# Autodesk Inventor assembly: BG200_trajan20_21
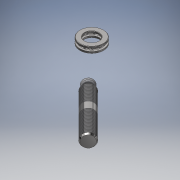
[picture p0: Inventor's stored thumbnail of the model, 180x180]
Saved by Autodesk Inventor 2022.2 (Build 262287000, 287)
## iProperties
Company: HTBLA Kaindorf
RuleStatus: InUse
Created: 2022-08-02
Part Number: BG200_trajan20_21
Project: Zeichenmaschine_v2
Material: Generisch
Description: rolle
Document SubType Name: Assembly
Designer: trajan20
AfterDocNew0: iProperties-Editor_aufrufen
Author: jan
Keywords: 2021
## Documents named in this file (5)
- C:\Users\jan\Documents\DrawMachine\DrawMachineConstruction\Projekt\Zeichenmaschine_v2\BG200_trajan20_21_Zeichenmaschine_v2_rolle.iam
- C:\Users\jan\Documents\DrawMachine\DrawMachineConstruction\Projekt\Zeichenmaschine_v2\BT105_trajan20_21_Zeichenmaschine_v2_halter final.ipt
- C:\Users\jan\Documents\DrawMachine\DrawMachineConstruction\Projekt\Zeichenmaschine_v2\BT101_trajan20_21_Zeichenmaschine_v2_rad.ipt
- C:\Users\jan\Documents\DrawMachine\DrawMachineConstruction\Projekt\Zeichenmaschine_v2\BG200_trajan20_21_Zeichenmaschine_v2_rolle\Konstruktions-Assistent\Lager1.iam
- C:\Users\jan\Documents\DrawMachine\DrawMachineConstruction\Projekt\Zeichenmaschine_v2\Normteile\de-DE\DIN 835\DIN 835 - M24 x 70 - 3.ipt
## Components (4 placed, 4 different names)
1. BT105_trajan20_21_Zeichenmaschine_v2_halter final:1 — Passend:1, Passend:2, Passend:3
2. BT101_trajan20_21_Zeichenmaschine_v2_rad:1 — Passend:1, Passend:2
3. DIN 835 M24 x 70:1 — Passend:3
4. Lager:1 [sub-assembly]
## Relationships (3: Mate 3)
- Passend:1 [Mate]: BT105_trajan20_21_Zeichenmaschine_v2_halter final:1 ↔ BT101_trajan20_21_Zeichenmaschine_v2_rad:1
- Passend:2 [Mate] (0.1 mm): BT105_trajan20_21_Zeichenmaschine_v2_halter final:1 ↔ BT101_trajan20_21_Zeichenmaschine_v2_rad:1
- Passend:3 [Mate]: BT105_trajan20_21_Zeichenmaschine_v2_halter final:1 ↔ DIN 835 M24 x 70:1
